# Autodesk Inventor assembly: Oberschenkel
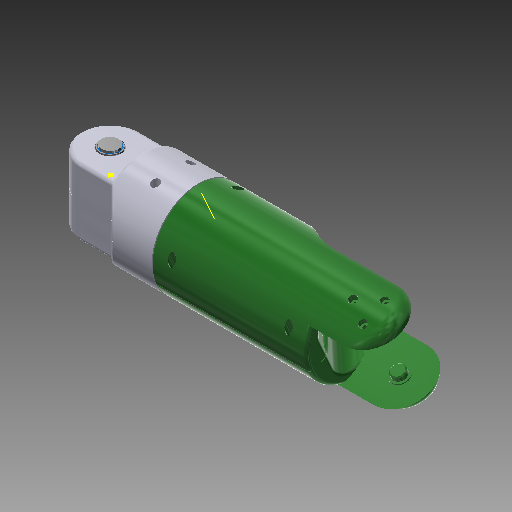
[picture p0: Inventor's stored thumbnail of the model, 512x512]
Saved by Autodesk Inventor 2018 (Build 220112000, 112)
## iProperties
Part Number: Oberschenkel
Material: Generisch
Document SubType Name: Assembly
Designer: Jochen Alt
Mass: 186.402 g
Surface Area: 1060.57 cm^2
Volume: 140.56 cm^3
Density: 1.32614 g/cm^3
Author: Jochen Alt
## Documents named in this file (10)
- D:\Projects\Manfred\cad\Inventor\Thigh.iam
- D:\Projects\Manfred\cad\Inventor\Thigh.ipt
- D:\Projects\Manfred\cad\Inventor\Thigh Bushing.ipt
- D:\Projects\Manfred\cad\Inventor\Herkulex DRS-010x\HerkuleX DRS-0101.iam
- D:\Projects\Manfred\cad\Inventor\Knee.ipt
- D:\Projects\Manfred\cad\Inventor\Oberschenkel\Konstruktions-Assistent\Kegelräder1.iam
- D:\Projects\Manfred\cad\Inventor\Herkulex DRS-010x\W 61707-2RS1.ipt
- D:\Projects\Manfred\cad\Inventor\Herkulex DRS-010x\HerkuleX DRS-0201.iam
- D:\Projects\Manfred\cad\Inventor\Rillenkugellager 11x7x3 inafag smr117.ipt
- D:\Projects\Manfred\cad\Inventor\Servobackaxis.ipt
## Components (10 placed, 9 different names)
1. Thigh Bushing:1 — Passend:30, Passend:31
2. HerkuleX DRS-0101:1 [sub-assembly] — Passend:28, Winkel:10, Passend:29
3. Knee:1 — Passend:26, Winkel:10, Passend:32
4. Kegelräder:2 [sub-assembly] — Passend:22, Passend:23, Winkel:9, Passend:26, Passend:28, Passend:29, Passend:41, Passend:42
5. W 61707-2RS1:1 — Passend:24, Passend:25, Passend:30, Passend:31
6. Thigh:1 — Passend:22, Passend:23, Winkel:9, Passend:24, Passend:25, Passend:32, Passend:33, Winkel:11, Passend:34, Passend:39
7. HerkuleX DRS-0201:1 [sub-assembly] — Passend:33, Winkel:11, Passend:34, Passend:40
8. Rillenkugellager 11x7x3 inafag smr117:1 — Passend:39, Passend:40, Passend:43, Passend:44
9. Rillenkugellager 11x7x3 inafag smr117:2 — Passend:41, Passend:42
10. Servobackaxis:1 — Passend:43, Passend:44
## Relationships (21: Mate 18, Angle 3)
- Passend:22 [Mate]: Kegelräder:2 ↔ Thigh:1
- Passend:23 [Mate]: Kegelräder:2 ↔ Thigh:1
- Winkel:9 [Angle] (0 deg): Kegelräder:2 ↔ Thigh:1
- Passend:24 [Mate]: W 61707-2RS1:1 ↔ Thigh:1
- Passend:25 [Mate] (0.1 mm): W 61707-2RS1:1 ↔ Thigh:1
- Passend:26 [Mate]: Knee:1 ↔ Kegelräder:2
- Passend:28 [Mate]: HerkuleX DRS-0101:1 ↔ Kegelräder:2
- Winkel:10 [Angle] (180 deg): HerkuleX DRS-0101:1 ↔ Knee:1
- Passend:29 [Mate]: HerkuleX DRS-0101:1 ↔ Kegelräder:2
- Passend:30 [Mate]: Thigh Bushing:1 ↔ W 61707-2RS1:1
- Passend:31 [Mate]: Thigh Bushing:1 ↔ W 61707-2RS1:1
- Passend:32 [Mate] (0.5 mm): Knee:1 ↔ Thigh:1
- Passend:33 [Mate]: Thigh:1 ↔ HerkuleX DRS-0201:1
- Winkel:11 [Angle] (90 deg): Thigh:1 ↔ HerkuleX DRS-0201:1
- Passend:34 [Mate] (0.1 mm): Thigh:1 ↔ HerkuleX DRS-0201:1
- Passend:39 [Mate]: Thigh:1 ↔ Rillenkugellager 11x7x3 inafag smr117:1
- Passend:40 [Mate] (0.5 mm): HerkuleX DRS-0201:1 ↔ Rillenkugellager 11x7x3 inafag smr117:1
- Passend:41 [Mate]: Kegelräder:2 ↔ Rillenkugellager 11x7x3 inafag smr117:2
- Passend:42 [Mate]: Kegelräder:2 ↔ Rillenkugellager 11x7x3 inafag smr117:2
- Passend:43 [Mate]: Rillenkugellager 11x7x3 inafag smr117:1 ↔ Servobackaxis:1
- Passend:44 [Mate]: Rillenkugellager 11x7x3 inafag smr117:1 ↔ Servobackaxis:1
